# Autodesk Inventor assembly: universal joint
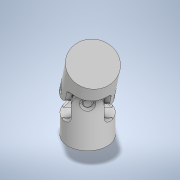
[picture p0: Inventor's stored thumbnail of the model, 180x180]
Saved by Autodesk Inventor 2022 (Build 260153000, 153)
## iProperties
Created: 2022-02-15
Part Number: universal joint
Document SubType Name: Assembly
Designer: RNG3nius
Author: RNG3nius
## Documents named in this file (4)
- D:\Mason\2021-2022\Capstone\Object Retrieval\universal joint.iam
- D:\Mason\2021-2022\Capstone\Object Retrieval\joint.ipt
- D:\Mason\2021-2022\Capstone\Object Retrieval\Nut.ipt
- D:\Mason\2021-2022\Capstone\Object Retrieval\shaft.ipt
## Components (7 placed, 3 different names)
1. Nut:1 — Mate:1, Mate:2
2. joint:1 — Rotational:1
3. joint:2 — Rotational:2
4. shaft:1 — Mate:1, Mate:2
5. shaft:2 — Rotational:1
6. shaft:3 — Rotational:2
7. shaft:4
## Component patterns: (4 elements, first: shaft:1)
## Relationships (4: Mate 2, RevoluteJoint 2)
- Mate:1: Nut:1 ↔ shaft:1
- Mate:2: Nut:1 ↔ shaft:1
- Rotational:1 [RevoluteJoint]: joint:1 ↔ shaft:2
- Rotational:2 [RevoluteJoint]: joint:2 ↔ shaft:3
